# Autodesk Inventor assembly: DeadWheelAssembly_MIR
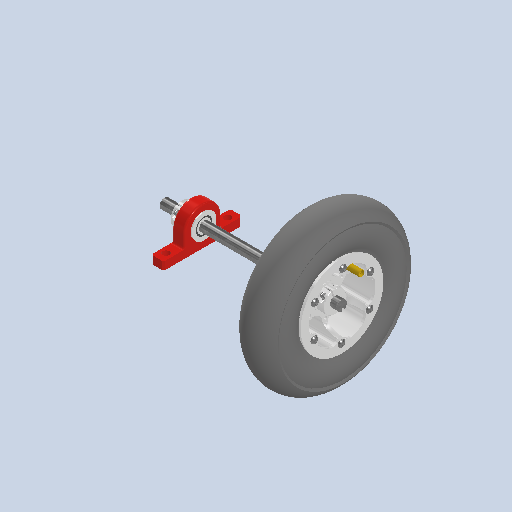
[picture p0: Inventor's stored thumbnail of the model, 512x512]
Saved by Autodesk Inventor 2023 (Build 270158000, 158)
## iProperties
Created: 2022-09-14
Part Number: DeadWheelAssembly_MIR
Document SubType Name: Assembly
Designer: PC
Author: PC
## Documents named in this file (6)
- C:\Users\PC\Documents\PersonalCAD\ARCIGVC\IGVC-Robot\DeadWheelAssembly_MIR.iam
- C:\Users\PC\Documents\PersonalCAD\ARCIGVC\IGVC-Robot\Bearing Housing_MIR2.ipt
- C:\Users\PC\Documents\PersonalCAD\ARCIGVC\IGVC-Robot\half in Bearing Flanged_MIR1.ipt
- C:\Users\PC\Documents\PersonalCAD\ARCIGVC\IGVC-Robot\8inPneumaticDEAD_MIR1.ipt
- C:\Users\PC\Documents\PersonalCAD\ARCIGVC\IGVC-Robot\SteelDeadAxel_MIR1.ipt
- C:\Users\PC\Documents\PersonalCAD\ARCIGVC\IGVC-Robot\am-2099 Collar Clamp, 0.5'' Bore, Aluminum_MIR1.ipt
## Components (12 placed, 5 different names)
1. Bearing Housing_MIR2:1 — Flush:2, Mate:1, Mate:6, Mate:5, Mate:7, Mate:3, Flush:3
2. Bearing Housing_MIR2:2 — Flush:2, Mate:1, Mate:9, Mate:2, Mate:8, Mate:4
3. half in Bearing Flanged_MIR1:1 — Mate:6, Mate:5, Mate:20
4. half in Bearing Flanged_MIR1:2 — Mate:9, Mate:2, Mate:15, Mate:14
5. half in Bearing Flanged_MIR1:3 — Mate:7, Mate:3
6. half in Bearing Flanged_MIR1:4 — Mate:8, Mate:4
7. 8inPneumaticDEAD_MIR1:1 — Mate:13, Mate:12, Mate:11, Mate:10, Flush:1
8. half in Bearing Flanged_MIR1:5 — Mate:13, Mate:12, Mate:16, Mate:18
9. half in Bearing Flanged_MIR1:6 — Mate:15, Mate:14, Mate:11, Mate:10
10. SteelDeadAxel_MIR1:1 — Flush:3, Mate:16, Flush:1, Mate:17, Mate:19
11. am-2099 Collar Clamp, 0.5'' Bore, Aluminum_MIR1:1 — Mate:18, Mate:17
12. am-2099 Collar Clamp, 0.5'' Bore, Aluminum_MIR1:2 — Mate:20, Mate:19
## Relationships (23: Mate 20, Flush 3)
- Flush:2: Bearing Housing_MIR2:1 ↔ Bearing Housing_MIR2:2
- Mate:1: Bearing Housing_MIR2:1 ↔ Bearing Housing_MIR2:2
- Mate:6: Bearing Housing_MIR2:1 ↔ half in Bearing Flanged_MIR1:1
- Mate:5: Bearing Housing_MIR2:1 ↔ half in Bearing Flanged_MIR1:1
- Mate:9: Bearing Housing_MIR2:2 ↔ half in Bearing Flanged_MIR1:2
- Mate:2: Bearing Housing_MIR2:2 ↔ half in Bearing Flanged_MIR1:2
- Mate:7: Bearing Housing_MIR2:1 ↔ half in Bearing Flanged_MIR1:3
- Mate:3: Bearing Housing_MIR2:1 ↔ half in Bearing Flanged_MIR1:3
- Mate:8: Bearing Housing_MIR2:2 ↔ half in Bearing Flanged_MIR1:4
- Mate:4: Bearing Housing_MIR2:2 ↔ half in Bearing Flanged_MIR1:4
- Mate:13: 8inPneumaticDEAD_MIR1:1 ↔ half in Bearing Flanged_MIR1:5
- Mate:12: 8inPneumaticDEAD_MIR1:1 ↔ half in Bearing Flanged_MIR1:5
- Mate:15 (12.7 mm): half in Bearing Flanged_MIR1:2 ↔ half in Bearing Flanged_MIR1:6
- Mate:14: half in Bearing Flanged_MIR1:2 ↔ half in Bearing Flanged_MIR1:6
- Mate:11: 8inPneumaticDEAD_MIR1:1 ↔ half in Bearing Flanged_MIR1:6
- Mate:10: 8inPneumaticDEAD_MIR1:1 ↔ half in Bearing Flanged_MIR1:6
- Flush:3 (33.655 mm): Bearing Housing_MIR2:1 ↔ SteelDeadAxel_MIR1:1
- Mate:16: half in Bearing Flanged_MIR1:5 ↔ SteelDeadAxel_MIR1:1
- Flush:1: 8inPneumaticDEAD_MIR1:1 ↔ SteelDeadAxel_MIR1:1
- Mate:18: half in Bearing Flanged_MIR1:5 ↔ am-2099 Collar Clamp, 0.5'' Bore, Aluminum_MIR1:1
- Mate:17: SteelDeadAxel_MIR1:1 ↔ am-2099 Collar Clamp, 0.5'' Bore, Aluminum_MIR1:1
- Mate:20: half in Bearing Flanged_MIR1:1 ↔ am-2099 Collar Clamp, 0.5'' Bore, Aluminum_MIR1:2
- Mate:19: SteelDeadAxel_MIR1:1 ↔ am-2099 Collar Clamp, 0.5'' Bore, Aluminum_MIR1:2
